# Autodesk Inventor assembly: Assembly1
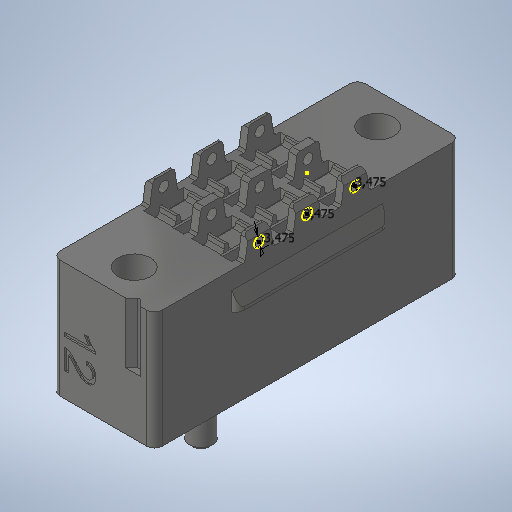
[picture p0: Inventor's stored thumbnail of the model, 512x512]
Saved by Autodesk Inventor 2025.1 (Build 291241000, 241)
## iProperties
Created: 2025-02-18
Part Number: Assembly1
Document SubType Name: Assembly
Designer: santiago
Author: santiago
## Documents named in this file (3)
- C:\Users\santiago\Documents\Tesis\3d models\scaled\Braille_assembly.iam
- C:\Users\santiago\Documents\Tesis\3d models\scaled\lower.ipt
- C:\Users\santiago\Documents\Tesis\3d models\scaled\Electromagnet.ipt
## Components (2 placed, 2 different names)
1. lower:1 — Insert:1
2. Electromagnet:1 — Insert:1
## Relationships (1: Insert 1)
- Insert:1: lower:1 ↔ Electromagnet:1
